# Autodesk Inventor assembly: 0313_KickerMount
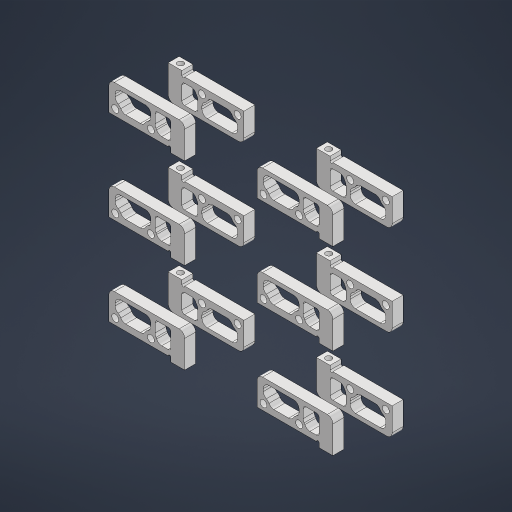
[picture p0: Inventor's stored thumbnail of the model, 512x512]
Saved by Autodesk Inventor 2024.2 (Build 282272000, 272)
## iProperties
Created: 2024-03-13
Part Number: 0313_KickerMount
Document SubType Name: Assembly
Designer: Hanaoka
Author: Hanaoka
## Documents named in this file (2)
- G:\共有ドライブ\reRo\05_個人\hanaoka\inventor\CAMpath\0313_KickerMount.iam
- G:\共有ドライブ\reRo\05_個人\hanaoka\inventor\KickerUnit\SolenoidMount.ipt
## Components (12 placed, 1 different names)
1. SolenoidMount:1 — メイト:1, メイト:2, メイト:3, メイト:4, メイト:5
2. SolenoidMount:2 — メイト:4, メイト:5, メイト:6
3. SolenoidMount:3
4. SolenoidMount:4
5. SolenoidMount:5
6. SolenoidMount:6
7. SolenoidMount:7
8. SolenoidMount:8
9. SolenoidMount:9
10. SolenoidMount:10
11. SolenoidMount:11
12. SolenoidMount:12
## Component patterns: (6 elements, first: SolenoidMount:1 + SolenoidMount:2)
## Relationships (6: Mate 6)
- メイト:1 [Mate]: SolenoidMount:1
- メイト:2 [Mate]: SolenoidMount:1
- メイト:3 [Mate]: SolenoidMount:1
- メイト:4 [Mate] (4 mm): SolenoidMount:1 ↔ SolenoidMount:2
- メイト:5 [Mate] (4 mm): SolenoidMount:1 ↔ SolenoidMount:2
- メイト:6 [Mate]: SolenoidMount:2
